# Autodesk Inventor assembly: ASY TZS FDS way3
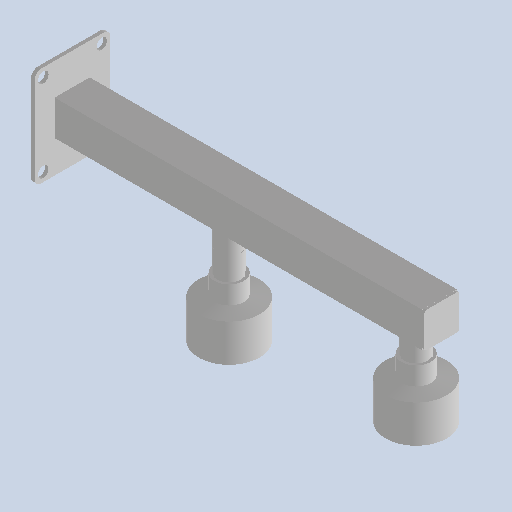
[picture p0: Inventor's stored thumbnail of the model, 512x512]
Saved by Autodesk Inventor 2025 (Build 290162010, 162A)
## iProperties
Created: 2025-07-02
Part Number: ASY TZS FDS way3
Document SubType Name: Assembly
Designer: user
Author: user
## Documents named in this file (7)
- C:\Users\pokla\Documents\Inventor\TZS-Tazovskiy\Filter D940\FDS 940\ASY TZS FDS way3.iam
- C:\Users\pokla\Documents\Inventor\TZS-Tazovskiy\Filter D940\FDS 940\TZS 756 FDS 940 way tube 3.ipt
- C:\Users\pokla\Documents\Inventor\TZS-Tazovskiy\Filter D940\FDS 940\TZS dummy filter element.ipt
- C:\Users\pokla\Documents\Inventor\TZS-Tazovskiy\Filter D940\FDS 940\TZS dummy pipe nippel.ipt
- C:\Users\pokla\Documents\Inventor\TZS-Tazovskiy\Filter D940\FDS 940\TZS 1757 FDS 940 way tube 7.ipt
- C:\Users\pokla\Documents\Inventor\TZS-Tazovskiy\Filter D940\FDS 940\TZS 760 FDS 940 FLANGE 3.ipt
- C:\Users\pokla\Documents\Inventor\TZS-Tazovskiy\Filter D940\FDS 940\TZS 766 FDS 940 CUP 1.ipt
## Components (8 placed, 6 different names)
1. TZS 756 FDS 1200 way tube 3.ipt:1 — Rigid:7
2. TZS dummy filter element.ipt:1
3. TZS dummy pipe nippel.ipt:1
4. TZS 1757 FDS 1200 way tube 7.ipt:1
5. TZS dummy filter element.ipt:2
6. TZS dummy pipe nippel.ipt:2
7. TZS 760 FDS 1200 FLANGE 3.ipt:1
8. TZS 766 FDS 1200 CUP 1.ipt:1 — Rigid:7
## Relationships (7: WeldJoint 7)
- [WeldJoint]: TZS dummy filter element.ipt:1 ↔ TZS dummy pipe nippel.ipt:1
- [WeldJoint]: TZS 756 FDS 1200 way tube 3.ipt:1 ↔ TZS dummy pipe nippel.ipt:1
- [WeldJoint]: TZS dummy filter element.ipt:2 ↔ TZS dummy pipe nippel.ipt:2
- [WeldJoint]: TZS 1757 FDS 1200 way tube 7.ipt:1 ↔ TZS dummy pipe nippel.ipt:2
- [WeldJoint]: TZS 756 FDS 1200 way tube 3.ipt:1 ↔ TZS 1757 FDS 1200 way tube 7.ipt:1
- [WeldJoint] (-3 mm): TZS 756 FDS 1200 way tube 3.ipt:1 ↔ TZS 760 FDS 1200 FLANGE 3.ipt:1
- Rigid:7 [WeldJoint]: TZS 756 FDS 1200 way tube 3.ipt:1 ↔ TZS 766 FDS 1200 CUP 1.ipt:1
## Named parameters: d34_d31 = 0 mm, d45_d43_d40_d37_d34_d31 = 0 mm
